# Autodesk Inventor assembly: fc16-079
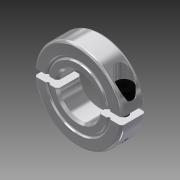
[picture p0: Inventor's stored thumbnail of the model, 180x180]
Saved by Autodesk Inventor 2016 SP1 (Build 200210100, 210)
## iProperties
Category: Shaft Collar
Company: Autodesk Inc.
Created: 2015-12-03
Part Number: fc16-079
Document SubType Name: Assembly
Designer: Autodesk Inc.
Catalog Web Link: http://www.ruland.com/shaft-collar.php?recordID=ENSP20-6-A
Vendor: Ruland
Author: Autodesk Inc.
Keywords: FIRSTChoice
## Documents named in this file (3)
- D:\FIRST\FRC KOP 2016\FRC FIRSTChoice 2016\fc16-079_ShaftCollar.iam
- D:\FIRST\FRC KOP 2016\FRC FIRSTChoice 2016\Parts\MISC_Collar_ENSP20-6-A.ipt
- D:\FIRST\FRC KOP 2016\FRC FIRSTChoice 2016\Parts\ISO 4762 - M2 x 6ISO.ipt
## Components (3 placed, 2 different names)
1. MISC_Collar_ENSP20-6-A:1 — Insert:1, Insert:2
2. ISO 4762 M2 x 6:1 — Insert:1
3. ISO 4762 M2 x 6:2 — Insert:2
## Relationships (2: Insert 2)
- Insert:1: MISC_Collar_ENSP20-6-A:1 ↔ ISO 4762 M2 x 6:1
- Insert:2: MISC_Collar_ENSP20-6-A:1 ↔ ISO 4762 M2 x 6:2
